# Autodesk Inventor assembly: TOLERANCE CALCULATOR
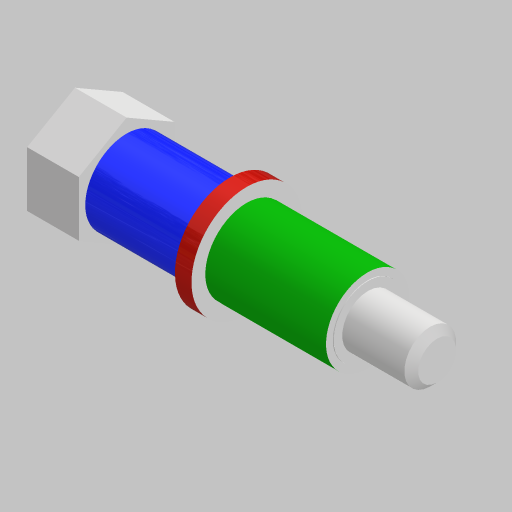
[picture p0: Inventor's stored thumbnail of the model, 512x512]
Saved by Autodesk Inventor 2024 (Build 280153000, 153)
## iProperties
Created: 2023-04-17
Part Number: TOLERANCE CALCULATOR
Document SubType Name: Assembly
Designer: rodar
Author: rodar
## Documents named in this file (5)
- C:\Users\arviau\Downloads\TOLERANCE CALCULATOR.iam
- G:\Unidades compartidas\Cursos de Ingeniería Mecánica UVG\Cursos IMXXX\IM3027 Introducción a Diseño y Manufactura CAD CAM\Clases - 2do semestre 2023\S13C2 - ACUMULACION DE TOLERANCIAS\Perno.ipt
- G:\Unidades compartidas\Cursos de Ingeniería Mecánica UVG\Cursos IMXXX\IM3027 Introducción a Diseño y Manufactura CAD CAM\Clases - 2do semestre 2023\S13C2 - ACUMULACION DE TOLERANCIAS\Buje azul.ipt
- G:\Unidades compartidas\Cursos de Ingeniería Mecánica UVG\Cursos IMXXX\IM3027 Introducción a Diseño y Manufactura CAD CAM\Clases - 2do semestre 2023\S13C2 - ACUMULACION DE TOLERANCIAS\Arandela.ipt
- G:\Unidades compartidas\Cursos de Ingeniería Mecánica UVG\Cursos IMXXX\IM3027 Introducción a Diseño y Manufactura CAD CAM\Clases - 2do semestre 2023\S13C2 - ACUMULACION DE TOLERANCIAS\Buje verde.ipt
## Components (4 placed, 4 different names)
1. Perno:1 — Flush:1
2. Buje azul:1 — Flush:1, Flush:2
3. Arandela:1 — Flush:2, Flush:3
4. Buje verde:1 — Flush:3
## Relationships (3: Flush 3)
- Flush:1: Perno:1 ↔ Buje azul:1
- Flush:2: Buje azul:1 ↔ Arandela:1
- Flush:3: Arandela:1 ↔ Buje verde:1
